# Autodesk Inventor assembly: Printer
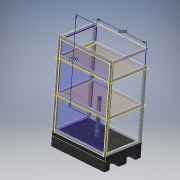
[picture p0: Inventor's stored thumbnail of the model, 180x180]
Saved by Autodesk Inventor 2016 (Build 200138000, 138)
## iProperties
Created: 2015-07-31
Part Number: Printer
Document SubType Name: Assembly
Designer: myhome
Author: myhome
## Documents named in this file (5)
- C:\Users\myhome\Documents\Inventor\Printer\Printer.iam
- C:\Users\myhome\Documents\Inventor\Printer\EpoxyGraniteBase\Base.iam
- C:\Users\myhome\Documents\Inventor\Printer\LinearActuator\RS-170435-1.iam
- C:\Users\myhome\Documents\Inventor\Printer\FrameExtruded\Frame.iam
- Printer.iam
## Components (3 placed, 3 different names)
1. Base:1 [sub-assembly] — Planar:1, Rigid:1
2. RS-170435-1:1 [sub-assembly] — Planar:1
3. Printer:1 [sub-assembly] — Rigid:1
## Relationships (2: PlanarJoint 1, WeldJoint 1)
- Planar:1: Base:1 ↔ RS-170435-1:1
- Rigid:1 [WeldJoint]: Base:1 ↔ Printer:1
